# Autodesk Inventor assembly: z_assembly
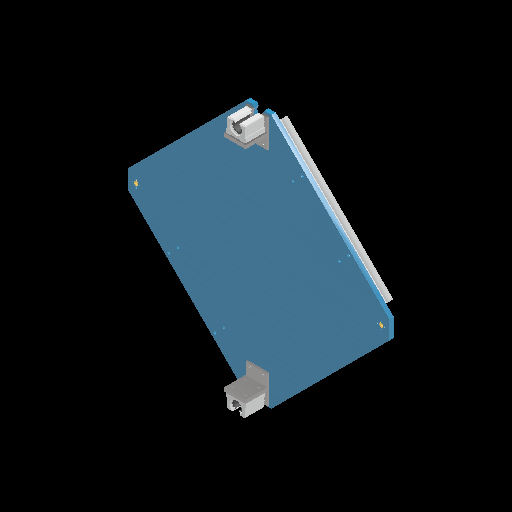
[picture p0: Inventor's stored thumbnail of the model, 512x512]
Saved by Autodesk Inventor 2026.1 (Build 301233000, 233)
## iProperties
Created: 2025-09-21
Part Number: z_assembly
Document SubType Name: Assembly
Designer: drago
Author: drago
## Documents named in this file (6)
- C:\Users\drago\Desktop\_QIST4500_Multidisciplinary_Team_Project\Proteox MX magnet positioner CAD\z_plate\z_assembly.iam
- C:\Users\drago\Desktop\_QIST4500_Multidisciplinary_Team_Project\Proteox MX magnet positioner CAD\z_plate\z_plate.ipt
- C:\Users\drago\Desktop\_QIST4500_Multidisciplinary_Team_Project\Proteox MX magnet positioner CAD\z_plate\SBR16UU_zBracket.ipt
- C:\Users\drago\Desktop\_QIST4500_Multidisciplinary_Team_Project\Proteox MX magnet positioner CAD\z_plate\Trapezoidal lead screw Nut tr8x8-4.ipt
- C:\Users\drago\Desktop\_QIST4500_Multidisciplinary_Team_Project\Proteox MX magnet positioner CAD\z_plate\SBR16UU.ipt
- C:\Users\drago\Desktop\_QIST4500_Multidisciplinary_Team_Project\Proteox MX magnet positioner CAD\z_plate\rail.ipt
## Components (9 placed, 5 different names)
1. z_plate:1 — Mate:21, Mate:22, Mate:23, Mate:24, Mate:25, Mate:26, Mate:27, Mate:28, Mate:29, Mate:30, Mate:31, Mate:32, Mate:33, Mate:34, Mate:41, Mate:42, Mate:43, Mate:44, Mate:45, Mate:46
2. SBR16UU_zBracket:1 — Mate:26, Mate:27, Mate:28, Mate:38, Mate:39, Mate:40
3. SBR16UU_zBracket:2 — Mate:23, Mate:24, Mate:25, Mate:35, Mate:36, Mate:37
4. SBR16UU:1 — Mate:35, Mate:36, Mate:37
5. SBR16UU:2 — Mate:38, Mate:39, Mate:40
6. Trapezoidal lead screw Nut tr8x8-4:1 — Mate:32, Mate:33, Mate:34
7. Trapezoidal lead screw Nut tr8x8-4:2 — Mate:29, Mate:30, Mate:31
8. rail:1 — Mate:41, Mate:45, Mate:46
9. rail:2 — Mate:42, Mate:43, Mate:44
## Relationships (26: Mate 26)
- Mate:21: z_plate:1
- Mate:22: z_plate:1
- Mate:23: z_plate:1 ↔ SBR16UU_zBracket:2
- Mate:24: z_plate:1 ↔ SBR16UU_zBracket:2
- Mate:25: z_plate:1 ↔ SBR16UU_zBracket:2
- Mate:26: z_plate:1 ↔ SBR16UU_zBracket:1
- Mate:27: z_plate:1 ↔ SBR16UU_zBracket:1
- Mate:28: z_plate:1 ↔ SBR16UU_zBracket:1
- Mate:29: z_plate:1 ↔ Trapezoidal lead screw Nut tr8x8-4:2
- Mate:30: z_plate:1 ↔ Trapezoidal lead screw Nut tr8x8-4:2
- Mate:31: z_plate:1 ↔ Trapezoidal lead screw Nut tr8x8-4:2
- Mate:32: z_plate:1 ↔ Trapezoidal lead screw Nut tr8x8-4:1
- Mate:33: z_plate:1 ↔ Trapezoidal lead screw Nut tr8x8-4:1
- Mate:34: z_plate:1 ↔ Trapezoidal lead screw Nut tr8x8-4:1
- Mate:35: SBR16UU_zBracket:2 ↔ SBR16UU:1
- Mate:36: SBR16UU_zBracket:2 ↔ SBR16UU:1
- Mate:37: SBR16UU_zBracket:2 ↔ SBR16UU:1
- Mate:38: SBR16UU_zBracket:1 ↔ SBR16UU:2
- Mate:39: SBR16UU_zBracket:1 ↔ SBR16UU:2
- Mate:40: SBR16UU_zBracket:1 ↔ SBR16UU:2
- Mate:41: z_plate:1 ↔ rail:1
- Mate:42: z_plate:1 ↔ rail:2
- Mate:43: z_plate:1 ↔ rail:2
- Mate:44: z_plate:1 ↔ rail:2
- Mate:45: z_plate:1 ↔ rail:1
- Mate:46: z_plate:1 ↔ rail:1
